# Autodesk Inventor assembly: Assembly1
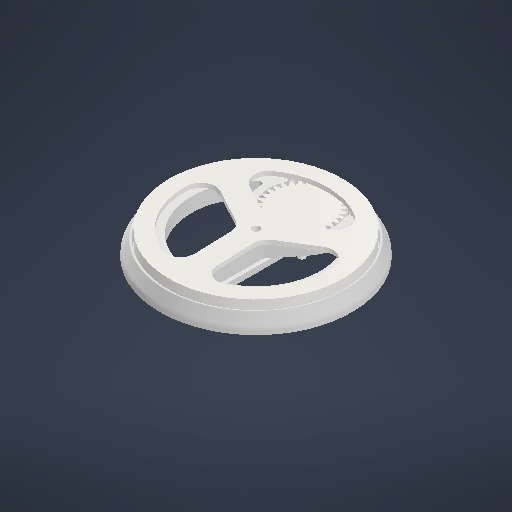
[picture p0: Inventor's stored thumbnail of the model, 512x512]
Saved by Autodesk Inventor 2026.2 (Build 302298000, 298)
## iProperties
Created: 2026-01-26
Part Number: Assembly1
Document SubType Name: Assembly
Designer: Cobble
Author: Cobble
## Documents named in this file (5)
- D:\CAD\Shot Filler V3\Assembly1.iam
- D:\CAD\Shot Filler V3\Gear Holder 1.ipt
- D:\CAD\Shot Filler V3\Gear Holder 2.ipt
- D:\CAD\Shot Filler V3\Assembly1\Design Accelerator\Spur Gear12.ipt
- D:\CAD\Shot Filler V3\Assembly1\Design Accelerator\Spur Gear22.ipt
## Components (4 placed, 4 different names)
1. Gear Holder 1:1 — Mate:3, Mate:4, Insert:4, Insert:5
2. Gear Holder 2:1 — Mate:3, Insert:3, Mate:4, Insert:4
3. Spur Gear1:1 — Rotation:1, Insert:3
4. Spur Gear2:1 — Rotation:1, Insert:5
## Relationships (6: Insert 3, Mate 2, RelateRotation 1)
- Mate:3: Gear Holder 1:1 ↔ Gear Holder 2:1
- Rotation:1 [RelateRotation] (2.4839 ul): Spur Gear1:1 ↔ Spur Gear2:1
- Insert:3: Gear Holder 2:1 ↔ Spur Gear1:1
- Mate:4: Gear Holder 1:1 ↔ Gear Holder 2:1
- Insert:4: Gear Holder 1:1 ↔ Gear Holder 2:1
- Insert:5: Gear Holder 1:1 ↔ Spur Gear2:1
